# Autodesk Inventor assembly: Robot
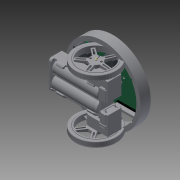
[picture p0: Inventor's stored thumbnail of the model, 180x180]
Saved by Autodesk Inventor 2014 (Build 180170000, 170)
## iProperties
Created: 2013-06-25
Part Number: Robot
Document SubType Name: Assembly
Designer: Felix
Author: Felix
## Documents named in this file (6)
- C:\Users\Felix\Desktop\Beep\Hardware\3D-CAD\Robot.iam
- C:\Users\Felix\Desktop\Beep\Hardware\3D-CAD\Pololu_gear_motor_1_180\gear_motor.iam
- C:\Users\Felix\Desktop\Beep\Hardware\3D-CAD\Pololu_Wheel_6mm\Wheel.iam
- C:\Users\Felix\Desktop\Beep\Hardware\3D-CAD\RaspberryPi\RaspberryPi_with_frame.iam
- C:\Users\Felix\Desktop\Beep\Hardware\3D-CAD\battery_holder\holder_with_batteries_18500.iam
- C:\Users\Felix\Desktop\Beep\Hardware\3D-CAD\battery_holder\holder_with_batteries_18650.iam
## Components (7 placed, 5 different names)
1. gear_motor:1 [sub-assembly] — Passend:1, Passend:5, Passend:6, Passend:7, Fluchtend:3, Passend:13, Passend:14, Passend:16, Passend:18, Passend:19
2. gear_motor:2 [sub-assembly] — Passend:1, Passend:2, Passend:3, Passend:4, Fluchtend:3, Fluchtend:4, Fluchtend:5, Passend:12, Passend:15
3. Wheel:1 [sub-assembly] — Passend:5, Passend:6, Passend:7
4. Wheel:2 [sub-assembly] — Passend:2, Passend:3, Passend:4
5. RaspberryPi_with_frame:1 [sub-assembly] — Passend:17
6. holder_with_batteries_18500:1 [sub-assembly] — Fluchtend:4, Passend:13, Passend:14, Passend:15, Passend:17
7. holder_with_batteries_18650:1 [sub-assembly] — Fluchtend:5, Passend:12, Passend:16
## Relationships (18: Mate 15, Flush 3)
- Passend:1 [Mate]: gear_motor:1 ↔ gear_motor:2
- Passend:2 [Mate]: gear_motor:2 ↔ Wheel:2
- Passend:3 [Mate]: gear_motor:2 ↔ Wheel:2
- Passend:4 [Mate]: gear_motor:2 ↔ Wheel:2
- Passend:5 [Mate]: gear_motor:1 ↔ Wheel:1
- Passend:6 [Mate]: gear_motor:1 ↔ Wheel:1
- Passend:7 [Mate]: gear_motor:1 ↔ Wheel:1
- Fluchtend:3 [Flush]: gear_motor:1 ↔ gear_motor:2
- Fluchtend:4 [Flush]: gear_motor:2 ↔ holder_with_batteries_18500:1
- Fluchtend:5 [Flush]: gear_motor:2 ↔ holder_with_batteries_18650:1
- Passend:12 [Mate]: gear_motor:2 ↔ holder_with_batteries_18650:1
- Passend:13 [Mate]: gear_motor:1 ↔ holder_with_batteries_18500:1
- Passend:14 [Mate]: gear_motor:1 ↔ holder_with_batteries_18500:1
- Passend:15 [Mate]: gear_motor:2 ↔ holder_with_batteries_18500:1
- Passend:16 [Mate]: gear_motor:1 ↔ holder_with_batteries_18650:1
- Passend:17 [Mate] (4 mm): RaspberryPi_with_frame:1 ↔ holder_with_batteries_18500:1
- Passend:18 [Mate]: gear_motor:1
- Passend:19 [Mate]: gear_motor:1
